# Autodesk Inventor assembly: CuvetteHolder
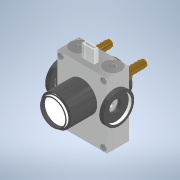
[picture p0: Inventor's stored thumbnail of the model, 180x180]
Saved by Autodesk Inventor 2022 (Build 260153000, 153)
## iProperties
Created: 2021-04-01
Part Number: CuvetteHolder
Document SubType Name: Assembly
Designer: wilso
Author: wilso
## Documents named in this file (14)
- D:\Dropbox\3D_Modeling\TemperatureControlledSampleHolder\CuvetteHolder.iam
- D:\Dropbox\3D_Modeling\TemperatureControlledSampleHolder\CuvetteHolderBody.ipt
- D:\Dropbox\3D_Modeling\TemperatureControlledSampleHolder\CuvetteHolderFace.ipt
- D:\Dropbox\3D_Modeling\TemperatureControlledSampleHolder\2mmCuvette.ipt
- D:\Dropbox\3D_Modeling\TemperatureControlledSampleHolder\91253A329_Black-Oxide Alloy Steel Hex Drive Flat Head Screw.ipt
- D:\Dropbox\3D_Modeling\TemperatureControlledSampleHolder\1075T49_Brass Barbed Hose Fitting for Air and Water.ipt
- D:\Dropbox\3D_Modeling\TemperatureControlledSampleHolder\34665K31_2017 Aluminum.ipt
- D:\Dropbox\3D_Modeling\TemperatureControlledSampleHolder\9657K261_Compression Spring.ipt
- D:\Dropbox\3D_Modeling\TemperatureControlledSampleHolder\91318A510_18-8 Stainless Steel Hollow-Lock Set Screws.ipt
- D:\Dropbox\3D_Modeling\TemperatureControlledSampleHolder\92949A132_18-8 Stainless Steel Button Head Hex Drive Screw.ipt
- D:\Dropbox\3D_Modeling\TemperatureControlledSampleHolder\SM1A1.ipt
- D:\Dropbox\3D_Modeling\TemperatureControlledSampleHolder\SM1AD18.ipt
- D:\Dropbox\3D_Modeling\TemperatureControlledSampleHolder\SM1L05.ipt
- D:\Dropbox\3D_Modeling\TemperatureControlledSampleHolder\SM1L10.ipt
## Components (20 placed, 13 different names)
1. CuvetteHolderBody:1 — Mate:1, Mate:2, Mate:3, Mate:5, Mate:6, Flush:2, Flush:3, Mate:10, Mate:11, Mate:12, Mate:13, Mate:14, Mate:15, Mate:16, Mate:17, Mate:18, Mate:19, Mate:20, Mate:22, Flush:4, Mate:31, Mate:32, Mate:33, Mate:34, Mate:39, Mate:40
2. CuvetteHolderFace:1 — Mate:1, Mate:2, Mate:3, Mate:4, Flush:1, Mate:23, Mate:24, Mate:25, Mate:26, Mate:27, Mate:28, Mate:29, Mate:30, Mate:36, Mate:37
3. 2mmCuvette:1 — Mate:4, Mate:5, Mate:6, Mate:21, Mate:35
4. 91253A329_Black-Oxide Alloy Steel Hex Drive Flat Head Screw:4 — Flush:3, Mate:15
5. 91253A329_Black-Oxide Alloy Steel Hex Drive Flat Head Screw:5 — Flush:2, Mate:14
6. 91253A329_Black-Oxide Alloy Steel Hex Drive Flat Head Screw:6 — Flush:1, Mate:16
7. 1075T49_Brass Barbed Hose Fitting for Air and Water:1 — Mate:10, Mate:13
8. 1075T49_Brass Barbed Hose Fitting for Air and Water:2 — Mate:11, Mate:12
9. 34665K31_2017 Aluminum:1 — Mate:20, Mate:21
10. 9657K261_Compression Spring:1
11. 91318A510_18-8 Stainless Steel Hollow-Lock Set Screws:1 — Mate:22, Flush:4
12. 92949A132_18-8 Stainless Steel Button Head Hex Drive Screw:1 — Mate:25, Mate:28
13. 92949A132_18-8 Stainless Steel Button Head Hex Drive Screw:2 — Mate:23, Mate:29
14. 92949A132_18-8 Stainless Steel Button Head Hex Drive Screw:3 — Mate:24, Mate:30
15. 92949A132_18-8 Stainless Steel Button Head Hex Drive Screw:4 — Mate:26, Mate:27
16. SM1A1:1 — Mate:31, Mate:33
17. SM1A1:2 — Mate:32, Mate:34
18. SM1AD18:1 — Mate:35, Mate:36, Mate:38
19. SM1L05:1 — Mate:39, Mate:40
20. SM1L10:1 — Mate:37, Mate:38
## Relationships (41: Mate 37, Flush 4)
- Mate:1 (0.1 mm): CuvetteHolderBody:1 ↔ CuvetteHolderFace:1
- Mate:2 (0.1 mm): CuvetteHolderBody:1 ↔ CuvetteHolderFace:1
- Mate:3 (0.1 mm): CuvetteHolderBody:1 ↔ CuvetteHolderFace:1
- Mate:4 (0.01 mm): CuvetteHolderFace:1 ↔ 2mmCuvette:1
- Mate:5 (0.1 mm): CuvetteHolderBody:1 ↔ 2mmCuvette:1
- Mate:6 (-5 mm): CuvetteHolderBody:1 ↔ 2mmCuvette:1
- Flush:1 (-0.1 mm): CuvetteHolderFace:1 ↔ 91253A329_Black-Oxide Alloy Steel Hex Drive Flat Head Screw:6
- Flush:2 (-0.1 mm): CuvetteHolderBody:1 ↔ 91253A329_Black-Oxide Alloy Steel Hex Drive Flat Head Screw:5
- Flush:3 (-0.1 mm): CuvetteHolderBody:1 ↔ 91253A329_Black-Oxide Alloy Steel Hex Drive Flat Head Screw:4
- Mate:10: CuvetteHolderBody:1 ↔ 1075T49_Brass Barbed Hose Fitting for Air and Water:1
- Mate:11: CuvetteHolderBody:1 ↔ 1075T49_Brass Barbed Hose Fitting for Air and Water:2
- Mate:12: CuvetteHolderBody:1 ↔ 1075T49_Brass Barbed Hose Fitting for Air and Water:2
- Mate:13: CuvetteHolderBody:1 ↔ 1075T49_Brass Barbed Hose Fitting for Air and Water:1
- Mate:14: CuvetteHolderBody:1 ↔ 91253A329_Black-Oxide Alloy Steel Hex Drive Flat Head Screw:5
- Mate:15: CuvetteHolderBody:1 ↔ 91253A329_Black-Oxide Alloy Steel Hex Drive Flat Head Screw:4
- Mate:16: CuvetteHolderBody:1 ↔ 91253A329_Black-Oxide Alloy Steel Hex Drive Flat Head Screw:6
- Mate:17: CuvetteHolderBody:1
- Mate:18: CuvetteHolderBody:1
- Mate:19: CuvetteHolderBody:1
- Mate:20: CuvetteHolderBody:1 ↔ 34665K31_2017 Aluminum:1
- Mate:21 (3.175 mm): 2mmCuvette:1 ↔ 34665K31_2017 Aluminum:1
- Mate:22: CuvetteHolderBody:1 ↔ 91318A510_18-8 Stainless Steel Hollow-Lock Set Screws:1
- Flush:4 (-1.5 mm): CuvetteHolderBody:1 ↔ 91318A510_18-8 Stainless Steel Hollow-Lock Set Screws:1
- Mate:23: CuvetteHolderFace:1 ↔ 92949A132_18-8 Stainless Steel Button Head Hex Drive Screw:2
- Mate:24: CuvetteHolderFace:1 ↔ 92949A132_18-8 Stainless Steel Button Head Hex Drive Screw:3
- Mate:25: CuvetteHolderFace:1 ↔ 92949A132_18-8 Stainless Steel Button Head Hex Drive Screw:1
- Mate:26: CuvetteHolderFace:1 ↔ 92949A132_18-8 Stainless Steel Button Head Hex Drive Screw:4
- Mate:27: CuvetteHolderFace:1 ↔ 92949A132_18-8 Stainless Steel Button Head Hex Drive Screw:4
- Mate:28: CuvetteHolderFace:1 ↔ 92949A132_18-8 Stainless Steel Button Head Hex Drive Screw:1
- Mate:29: CuvetteHolderFace:1 ↔ 92949A132_18-8 Stainless Steel Button Head Hex Drive Screw:2
- Mate:30: CuvetteHolderFace:1 ↔ 92949A132_18-8 Stainless Steel Button Head Hex Drive Screw:3
- Mate:31: CuvetteHolderBody:1 ↔ SM1A1:1
- Mate:32: CuvetteHolderBody:1 ↔ SM1A1:2
- Mate:33: CuvetteHolderBody:1 ↔ SM1A1:1
- Mate:34: CuvetteHolderBody:1 ↔ SM1A1:2
- Mate:35: 2mmCuvette:1 ↔ SM1AD18:1
- Mate:36: CuvetteHolderFace:1 ↔ SM1AD18:1
- Mate:37: CuvetteHolderFace:1 ↔ SM1L10:1
- Mate:38: SM1AD18:1 ↔ SM1L10:1
- Mate:39: CuvetteHolderBody:1 ↔ SM1L05:1
- Mate:40: CuvetteHolderBody:1 ↔ SM1L05:1
